# Autodesk Inventor assembly: Chain-Sprocket to Engine
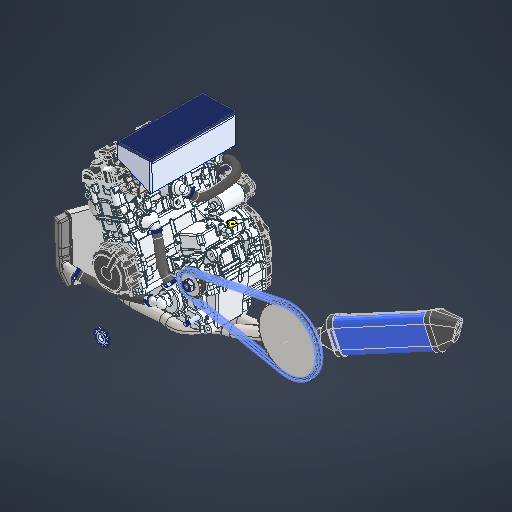
[picture p0: Inventor's stored thumbnail of the model, 512x512]
Saved by Autodesk Inventor 2027 (Build 310192000, 192)
## iProperties
Created: 2026-06-07
Part Number: Chain-Sprocket to Engine
Document SubType Name: Assembly
Designer: W Ahmad
Title: Chain-sprocket to engine
Author: W Ahmad
## Documents named in this file (2)
- C:\Users\W Ahmad\Desktop\FSAE- Summer 2026 Project\FSAE CAD\GOGO_KART_FSAE\Chain-Sprocket to Engine.iam
- C:\Users\W Ahmad\Desktop\FSAE- Summer 2026 Project\FSAE CAD\GOGO_KART_FSAE\2005-gsxr-600-engine-model-1.snapshot.2\Engine\Engine Assembly\Engine Assembly\Engine Assembly.iam
## Components (1 placed, 1 different names)
1. Engine Assembly:1 [sub-assembly] — Flush:1, Flush:2, Flush:3
## Relationships (3: Flush 3)
- Flush:1: Engine Assembly:1
- Flush:2: Engine Assembly:1
- Flush:3: Engine Assembly:1
